# Autodesk Inventor assembly: Katze
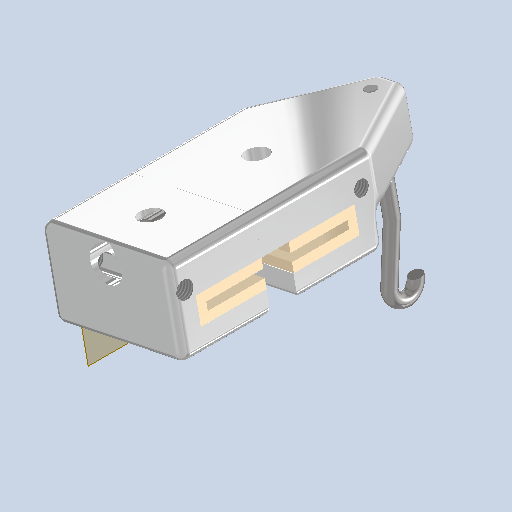
[picture p0: Inventor's stored thumbnail of the model, 512x512]
Saved by Autodesk Inventor 2025 (Build 290162010, 162A)
## iProperties
Created: 2024-11-19
Part Number: Katze
Document SubType Name: Assembly
Designer: Admin
Mass: 66.181 g
Surface Area: 161.129 cm^2
Volume: 25.2769 cm^3
Density: 2.61824 g/cm^3
Author: Admin
## Documents named in this file (10)
- C:\Users\Admin\GIT\HDVKBM\CAD\Krandemonstrator\Katze.iam
- C:\Users\Admin\GIT\HDVKBM\CAD\Krandemonstrator\Katze_Lagerhalter_hinten.ipt
- C:\Users\Admin\GIT\HDVKBM\CAD\Krandemonstrator\Katze_Lagerhalter_vorne.ipt
- C:\Users\Admin\GIT\HDVKBM\CAD\Krandemonstrator\LagerHH.ipt
- C:\Users\Admin\GIT\HDVKBM\CAD\Krandemonstrator\LagerHO.ipt
- C:\Users\Admin\GIT\HDVKBM\CAD\Krandemonstrator\M3 Haken 40mm.ipt
- C:\Users\Admin\Documents\Inventor\Content Center Files\R2025\de-DE\ISO 2338(1)\DIN EN ISO 2338 - 2 h8 x 10.ipt
- C:\Users\Admin\Documents\Inventor\Content Center Files\R2025\de-DE\ISO 4762(1)\DIN EN ISO 4762 - M4 x 12.ipt
- C:\Users\Admin\Documents\Inventor\Content Center Files\R2025\de-DE\ISO 2009(1)\ISO 2009 - M2 x 4 - DIN EN 2.ipt
- C:\Users\Admin\Documents\Inventor\Content Center Files\R2025\de-DE\ISO 4032(1)\ISO 4032 - M3DIN EN.ipt
## Components (19 placed, 9 different names)
1. Katze_Lagerhalter_hinten:1 — Starr:7, Starr:6, Planar:1, Planar:2, Planar:3, Planar:5
2. DIN EN ISO 2338 2 h8 x 10:1 — Starr:7, Zylindrisch:4
3. DIN EN ISO 2338 2 h8 x 10:2 — Starr:6, Zylindrisch:3
4. Katze_Lagerhalter_vorne:1 — Zylindrisch:3, Zylindrisch:4, Planar:7, Planar:8, Planar:10, Planar:12, Starr:13
5. DIN EN ISO 4762 M4 x 12:1
6. DIN EN ISO 2009 M2 x 4:1
7. DIN EN ISO 2009 M2 x 4:2
8. DIN EN ISO 2009 M2 x 4:3
9. DIN EN ISO 2009 M2 x 4:4
10. DIN EN ISO 2009 M2 x 4:5
11. DIN EN ISO 2009 M2 x 4:6
12. LagerHH:1 — Planar:1, Planar:2, Planar:4, Planar:6
13. LagerHH:2 — Planar:7, Planar:8, Planar:11, Planar:13
14. LagerHO:1 — Planar:10, Planar:11
15. LagerHO:2 — Planar:5, Planar:6
16. LagerHO:3 — Planar:3, Planar:4
17. LagerHO:4 — Planar:12, Planar:13
18. M3 Haken 40mm:1 — Starr:13
19. DIN EN 24032 M3:1
## Relationships (32: PlanarJoint 12, WeldJoint 10, CylindricalJoint 8, RevoluteJoint 1, Insert 1)
- Starr:7 [WeldJoint]: Katze_Lagerhalter_hinten:1 ↔ DIN EN ISO 2338 2 h8 x 10:1
- Starr:6 [WeldJoint]: Katze_Lagerhalter_hinten:1 ↔ DIN EN ISO 2338 2 h8 x 10:2
- Zylindrisch:3 [CylindricalJoint]: DIN EN ISO 2338 2 h8 x 10:2 ↔ Katze_Lagerhalter_vorne:1
- Zylindrisch:4 [CylindricalJoint]: DIN EN ISO 2338 2 h8 x 10:1 ↔ Katze_Lagerhalter_vorne:1
- [RevoluteJoint]: Katze_Lagerhalter_hinten:1 ↔ DIN EN ISO 4762 M4 x 12:1
- [WeldJoint] (0.165 mm): Katze_Lagerhalter_vorne:1 ↔ DIN EN ISO 4762 M4 x 12:1
- Planar:1: Katze_Lagerhalter_hinten:1 ↔ LagerHH:1
- [WeldJoint]: DIN EN ISO 2009 M2 x 4:1 ↔ LagerHH:1
- [CylindricalJoint]: Katze_Lagerhalter_hinten:1 ↔ DIN EN ISO 2009 M2 x 4:1
- Planar:2: Katze_Lagerhalter_hinten:1 ↔ LagerHH:1
- Planar:3: Katze_Lagerhalter_hinten:1 ↔ LagerHO:3
- [WeldJoint]: DIN EN ISO 2009 M2 x 4:5 ↔ LagerHO:3
- [CylindricalJoint]: Katze_Lagerhalter_hinten:1 ↔ DIN EN ISO 2009 M2 x 4:5
- Planar:4: LagerHH:1 ↔ LagerHO:3
- Planar:5: Katze_Lagerhalter_hinten:1 ↔ LagerHO:2
- [WeldJoint]: DIN EN ISO 2009 M2 x 4:4 ↔ LagerHO:2
- [CylindricalJoint]: Katze_Lagerhalter_hinten:1 ↔ DIN EN ISO 2009 M2 x 4:4
- Planar:6: LagerHH:1 ↔ LagerHO:2
- Planar:7: Katze_Lagerhalter_vorne:1 ↔ LagerHH:2
- [WeldJoint]: DIN EN ISO 2009 M2 x 4:6 ↔ LagerHH:2
- [CylindricalJoint]: Katze_Lagerhalter_vorne:1 ↔ DIN EN ISO 2009 M2 x 4:6
- Planar:8: Katze_Lagerhalter_vorne:1 ↔ LagerHH:2
- [WeldJoint]: DIN EN ISO 2009 M2 x 4:2 ↔ LagerHO:1
- Planar:10: Katze_Lagerhalter_vorne:1 ↔ LagerHO:1
- [CylindricalJoint]: Katze_Lagerhalter_vorne:1 ↔ DIN EN ISO 2009 M2 x 4:2
- Planar:11: LagerHH:2 ↔ LagerHO:1
- [WeldJoint]: DIN EN ISO 2009 M2 x 4:3 ↔ LagerHO:4
- Planar:12: Katze_Lagerhalter_vorne:1 ↔ LagerHO:4
- [CylindricalJoint]: Katze_Lagerhalter_vorne:1 ↔ DIN EN ISO 2009 M2 x 4:3
- Planar:13: LagerHH:2 ↔ LagerHO:4
- Starr:13 [WeldJoint]: Katze_Lagerhalter_vorne:1 ↔ M3 Haken 40mm:1
- [Insert]: Katze_Lagerhalter_vorne:1 ↔ DIN EN 24032 M3:1
